# Autodesk Inventor assembly: Assembly1
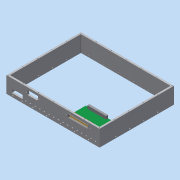
[picture p0: Inventor's stored thumbnail of the model, 180x180]
Saved by Autodesk Inventor 2016 (Build 200138000, 138)
## iProperties
Created: 2016-10-05
Part Number: Assembly1
Document SubType Name: Assembly
Designer: Zara
Author: Zara
## Documents named in this file (4)
- C:\Users\Zara\Documents\hera-cad\Node\SNAP V2 enclosure release - pack-n-go export\SNAP V2 enclosure release - pack-n-go export\Workspaces\Workspace\Assembly1.iam
- C:\Users\Zara\Documents\hera-cad\Node\SNAP V2 enclosure release - pack-n-go export\SNAP V2 enclosure release - pack-n-go export\Workspaces\Workspace\components\R58010-175-with SNAP V2 features.ipt
- R58010-175-with SNAP V2 features.ipt
- C:\Users\Zara\Documents\hera-cad\Node\mezzanineBoard.iam
## Components (2 placed, 2 different names)
1. R58010-175-with SNAP V2 features:1 — Flush:1, Mate:1, Mate:2
2. mezzanineBoard:1 [sub-assembly] — Flush:1, Mate:1, Mate:2
## Relationships (3: Mate 2, Flush 1)
- Flush:1 (6.477 mm): R58010-175-with SNAP V2 features:1 ↔ mezzanineBoard:1
- Mate:1 (27.6352 mm): R58010-175-with SNAP V2 features:1 ↔ mezzanineBoard:1
- Mate:2: R58010-175-with SNAP V2 features:1 ↔ mezzanineBoard:1
